# Autodesk Inventor assembly: odometery system assembly
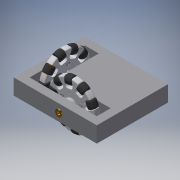
[picture p0: Inventor's stored thumbnail of the model, 180x180]
Saved by Autodesk Inventor 2019 (Build 230136000, 136)
## iProperties
Created: 2019-08-10
Part Number: odometery system assembly
Document SubType Name: Assembly
Designer: Delta
Author: Delta
## Documents named in this file (6)
- C:\Robotics\2019-20_CAD\offseason\random ideas\odometery system assembly.iam
- C:\Robotics\2019-20_CAD\3D Printer\odometery system base.ipt
- C:\Robotics\COTSParts\Tetrix\Bronze bushing.ipt
- C:\Robotics\COTSParts\Tetrix\Tetrix Hub - axle.ipt
- C:\Robotics\COTSParts\Tetrix\Tetrix Wheel 3 in omni.ipt
- C:\Robotics\COTSParts\Tetrix\Nylon spacer - small.ipt
## Components (11 placed, 5 different names)
1. odometery system base:1 — Mate:1, Mate:2, Mate:3, Mate:4, Mate:12, Mate:14, Mate:17, Mate:21
2. Bronze bushing:1 — Mate:1, Mate:2, Mate:11, Mate:18
3. Bronze bushing:2 — Mate:3, Mate:4, Mate:13, Mate:22
4. Tetrix Hub - axle:1 — Mate:8, Mate:9, Mate:10, Mate:13, Mate:14
5. Tetrix Hub - axle:2 — Mate:5, Mate:6, Mate:7, Mate:11, Mate:12
6. Tetrix Wheel 3 in omni:1 — Mate:5, Mate:6, Mate:7
7. Tetrix Wheel 3 in omni:2 — Mate:8, Mate:9, Mate:10
8. Nylon spacer - small:1 — Mate:19, Mate:20, Mate:21
9. Nylon spacer - small:2 — Mate:15, Mate:16, Mate:17
10. Nylon spacer - small:3 — Mate:19, Mate:20, Mate:22
11. Nylon spacer - small:4 — Mate:15, Mate:16, Mate:18
## Relationships (22: Mate 22)
- Mate:1: odometery system base:1 ↔ Bronze bushing:1
- Mate:2: odometery system base:1 ↔ Bronze bushing:1
- Mate:3: odometery system base:1 ↔ Bronze bushing:2
- Mate:4: odometery system base:1 ↔ Bronze bushing:2
- Mate:5: Tetrix Hub - axle:2 ↔ Tetrix Wheel 3 in omni:1
- Mate:6: Tetrix Hub - axle:2 ↔ Tetrix Wheel 3 in omni:1
- Mate:7: Tetrix Hub - axle:2 ↔ Tetrix Wheel 3 in omni:1
- Mate:8: Tetrix Hub - axle:1 ↔ Tetrix Wheel 3 in omni:2
- Mate:9: Tetrix Hub - axle:1 ↔ Tetrix Wheel 3 in omni:2
- Mate:10: Tetrix Hub - axle:1 ↔ Tetrix Wheel 3 in omni:2
- Mate:11: Bronze bushing:1 ↔ Tetrix Hub - axle:2
- Mate:12: odometery system base:1 ↔ Tetrix Hub - axle:2
- Mate:13: Bronze bushing:2 ↔ Tetrix Hub - axle:1
- Mate:14: odometery system base:1 ↔ Tetrix Hub - axle:1
- Mate:15: Nylon spacer - small:2 ↔ Nylon spacer - small:4
- Mate:16: Nylon spacer - small:2 ↔ Nylon spacer - small:4
- Mate:17: odometery system base:1 ↔ Nylon spacer - small:2
- Mate:18: Bronze bushing:1 ↔ Nylon spacer - small:4
- Mate:19: Nylon spacer - small:1 ↔ Nylon spacer - small:3
- Mate:20: Nylon spacer - small:1 ↔ Nylon spacer - small:3
- Mate:21: odometery system base:1 ↔ Nylon spacer - small:1
- Mate:22: Bronze bushing:2 ↔ Nylon spacer - small:3
